# Autodesk Inventor assembly: Tetrix_739275
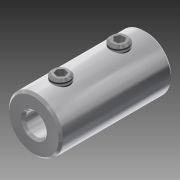
[picture p0: Inventor's stored thumbnail of the model, 180x180]
Saved by Autodesk Inventor 2016 SP1 (Build 200210100, 210)
## iProperties
Category: Fasteners and Hardware
Company: Autodesk Inc.
Created: 2014-11-27
Part Number: Tetrix_739275
Document SubType Name: Assembly
Designer: Tetrix
Catalog Web Link: http://www.tetrixrobotics.com/TETRIX_Axle_Shaft_Couplers
Vendor: Tetrix
Author: Autodesk Inc.
## Documents named in this file (3)
- D:\FIRST\FTC\FTC KOP 2016\Tetrix\Tetrix_739275.iam
- D:\FIRST\FTC\FTC KOP 2016\Tetrix\Tetrix_739275_Body.ipt
- D:\FIRST\FTC\FTC KOP 2016\Tetrix\Tetrix_739275_Screw.ipt
## Components (3 placed, 2 different names)
1. Tetrix_739275_Body:1 — Mate:1, Mate:2
2. Tetrix_739275_Screw:1 — Mate:1, Flush:1
3. Tetrix_739275_Screw:2 — Mate:2, Flush:1
## Relationships (3: Mate 2, Flush 1)
- Mate:1: Tetrix_739275_Body:1 ↔ Tetrix_739275_Screw:1
- Mate:2: Tetrix_739275_Body:1 ↔ Tetrix_739275_Screw:2
- Flush:1: Tetrix_739275_Screw:1 ↔ Tetrix_739275_Screw:2
